# Autodesk Inventor assembly: Sestava2
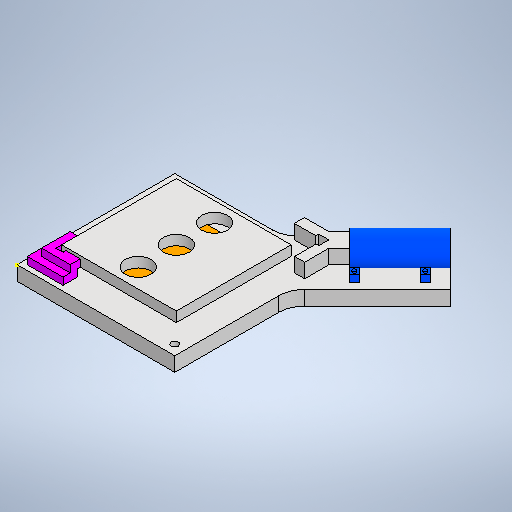
[picture p0: Inventor's stored thumbnail of the model, 512x512]
Saved by Autodesk Inventor 2025 (Build 290162000, 162)
## iProperties
Created: 2025-05-08
Part Number: Sestava2
Document SubType Name: Assembly
Designer: zdene
Mass: 232.884 g
Surface Area: 561.853 cm^2
Volume: 232.884 cm^3
Density: 1 g/cm^3
Author: zdene
## Documents named in this file (3)
- C:\Users\zdene\Desktop\Sestava2.iam
- C:\Users\zdene\Desktop\Součást1.ipt
- C:\Users\zdene\Desktop\Součást3.ipt
## Components (2 placed, 2 different names)
1. Součást1:1 — Proti sobě:1
2. Součást3:1 — Proti sobě:1
## Relationships (1: Mate 1)
- Proti sobě:1 [Mate]: Součást1:1 ↔ Součást3:1
